# Autodesk Inventor assembly: Fan_60x60x15
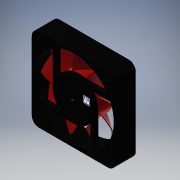
[picture p0: Inventor's stored thumbnail of the model, 180x180]
Saved by Autodesk Inventor 2017 (Build 210142000, 142)
## iProperties
Created: 2017-04-04
Part Number: Fan_60x60x15
Document SubType Name: Assembly
Designer: Edimay Prime
Author: Edimay Prime
## Documents named in this file (3)
- C:\Users\Edimay Prime\Documents\Fan_60x60x15.iam
- C:\Users\Edimay Prime\Documents\fan_chase_60.ipt
- C:\Users\Edimay Prime\Documents\Fan_rotor_60.ipt
## Components (2 placed, 2 different names)
1. fan_chase_60:1 — Insert:1
2. Fan_rotor_60:1 — Insert:1
## Relationships (1: Insert 1)
- Insert:1 (1 mm): fan_chase_60:1 ↔ Fan_rotor_60:1
